# Autodesk Inventor assembly: zlozenie_Z
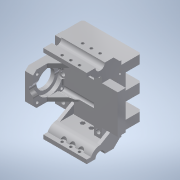
[picture p0: Inventor's stored thumbnail of the model, 180x180]
Saved by Autodesk Inventor 2020 (Build 240168000, 168)
## iProperties
Created: 2020-08-11
Part Number: zlozenie_Z
Material: Ogólny
Document SubType Name: Assembly
Designer: invin
Mass: 277.94 g
Surface Area: 715.515 cm^2
Volume: 180.364 cm^3
Density: 1.541 g/cm^3
Author: invin
## Documents named in this file (5)
- D:\KONIECTEGOKOŁCHOZU\MGR\model\Workspaces\Obszar roboczy\Assembly\Y\zlozenie_Z.iam
- D:\KONIECTEGOKOŁCHOZU\MGR\model\Workspaces\Obszar roboczy\Assembly\Y\ZY_mount.ipt
- D:\KONIECTEGOKOŁCHOZU\MGR\model\Workspaces\Obszar roboczy\OLD\ZY_rod_mount.ipt
- D:\KONIECTEGOKOŁCHOZU\MGR\model\Workspaces\Obszar roboczy\OLD\motormount.ipt
- D:\KONIECTEGOKOŁCHOZU\MGR\model\Workspaces\Obszar roboczy\Assembly\Z\Z_endstop_mount.ipt
## Components (4 placed, 4 different names)
1. ZY_mount:1 — Zestawiający:4, Zestawiający:5, Zestawiający:12, Równoległe:1, Równoległe:2, Zestawiające:13
2. ZY_rod_mount:1 — Zestawiający:4, Zestawiający:5, Zestawiający:9, Zestawiający:10, Zestawiający:11, Zestawiający:12
3. motormount:1 — Zestawiający:9, Zestawiający:10, Zestawiający:11, Zestawiające:14, Zestawiające:15, Zestawiające:16
4. Z_endstop_mount:1 — Zestawiające:14, Zestawiające:15, Zestawiające:16
## Relationships (12: Mate 10, Flush 2)
- Zestawiający:4 [Mate]: ZY_mount:1 ↔ ZY_rod_mount:1
- Zestawiający:5 [Mate]: ZY_mount:1 ↔ ZY_rod_mount:1
- Zestawiający:9 [Mate]: ZY_rod_mount:1 ↔ motormount:1
- Zestawiający:10 [Mate]: ZY_rod_mount:1 ↔ motormount:1
- Zestawiający:11 [Mate]: ZY_rod_mount:1 ↔ motormount:1
- Zestawiający:12 [Mate]: ZY_mount:1 ↔ ZY_rod_mount:1
- Równoległe:1 [Flush]: ZY_mount:1
- Równoległe:2 [Flush]: ZY_mount:1
- Zestawiające:13 [Mate]: ZY_mount:1
- Zestawiające:14 [Mate]: motormount:1 ↔ Z_endstop_mount:1
- Zestawiające:15 [Mate]: motormount:1 ↔ Z_endstop_mount:1
- Zestawiające:16 [Mate]: motormount:1 ↔ Z_endstop_mount:1
